# Autodesk Inventor assembly: !Conveyer
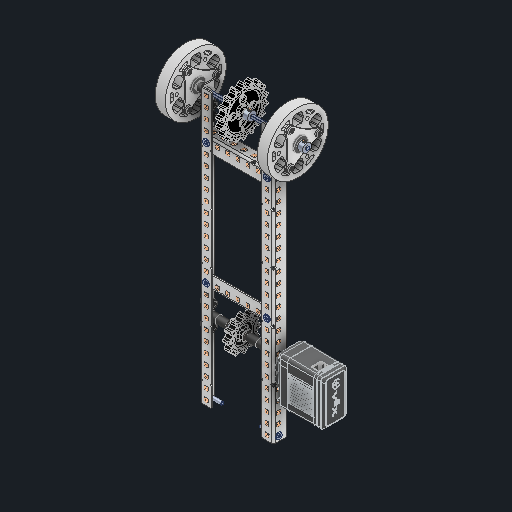
[picture p0: Inventor's stored thumbnail of the model, 512x512]
Saved by Autodesk Inventor 2025 (Build 290162000, 162)
## iProperties
Created: 2024-12-25
Part Number: !Conveyer
Document SubType Name: Assembly
Designer: Averey Ku
Author: Averey Ku
## Documents named in this file (4)
- D:\VEX\High Stakes\CAD\V4\Conveyer\!Conveyer.iam
- D:\VEX\High Stakes\CAD\V4\Conveyer\Structure.iam
- D:\VEX\High Stakes\CAD\V4\Conveyer\Bottom Roller.iam
- D:\VEX\High Stakes\CAD\V4\Conveyer\Top Roller.iam
## Components (3 placed, 3 different names)
1. Structure:1 [sub-assembly] — Insert:1, Mate:1
2. Bottom Roller:1 [sub-assembly] — Flush:1, Mate:1
3. Top Roller:1 [sub-assembly] — Insert:1, Flush:1
## Relationships (3: Insert 1, Flush 1, Mate 1)
- Insert:1: Structure:1 ↔ Top Roller:1
- Flush:1: Bottom Roller:1 ↔ Top Roller:1
- Mate:1: Structure:1 ↔ Bottom Roller:1
